# Autodesk Inventor assembly: Final Assembly
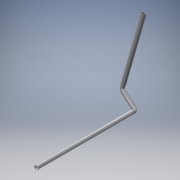
[picture p0: Inventor's stored thumbnail of the model, 180x180]
Saved by Autodesk Inventor 2018 (Build 220112000, 112)
## iProperties
Created: 2018-05-07
Part Number: Final Assembly
Document SubType Name: Assembly
Designer: 232963
Author: 232963
## Documents named in this file (6)
- P:\IED\SchoolCAD\Design Challenge\Final Assembly.iam
- P:\IED\SchoolCAD\Design Challenge\Main Rod.ipt
- P:\IED\SchoolCAD\Design Challenge\Short ROd.ipt
- P:\IED\SchoolCAD\Design Challenge\Slanted rod.ipt
- P:\IED\SchoolCAD\Design Challenge\real joint assemly.iam
- P:\IED\SchoolCAD\Design Challenge\Real Joint assembly 57d.iam
## Components (5 placed, 5 different names)
1. Main Rod:1 — Insert:1
2. Short ROd:1 — Insert:2, Insert:3
3. Slanted rod:1 — Insert:4
4. real joint assemly:1 [sub-assembly] — Insert:1, Insert:2
5. Real Joint assembly 57d:1 [sub-assembly] — Insert:3, Insert:4
## Relationships (4: Insert 4)
- Insert:1 (-12.7 mm): Main Rod:1 ↔ real joint assemly:1
- Insert:2 (-12.7 mm): Short ROd:1 ↔ real joint assemly:1
- Insert:3 (-12.7 mm): Short ROd:1 ↔ Real Joint assembly 57d:1
- Insert:4 (-12.7 mm): Slanted rod:1 ↔ Real Joint assembly 57d:1
